# Autodesk Inventor assembly: Print_Assembly_H0_NEM363
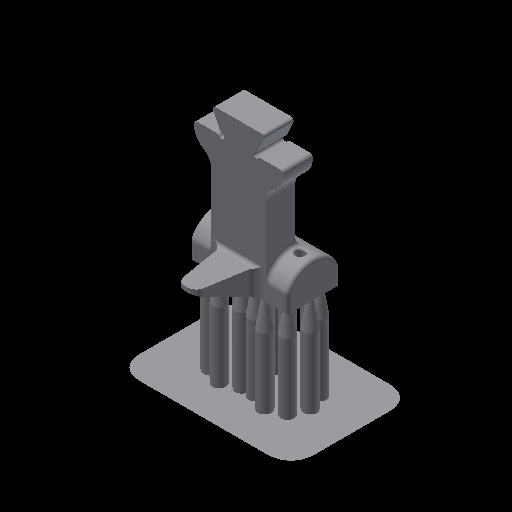
[picture p0: Inventor's stored thumbnail of the model, 512x512]
Saved by Autodesk Inventor 2026.2 (Build 302298010, 298A)
## iProperties
Manager: MANUTENÇÃO GUIFÕES - CP
Company: CP
Created: 2025-09-03
Part Number: Print_Assembly_H0_NEM363
Project: 0.00 0000/00
Checked By: PMFIGUEIREDO
Engr Approved By: JSSILVA
Description: NOME DA PEÇA/MONTAGEM
Document SubType Name: Assembly
Designer: TPMIRANDA
Engineer: ISO 2768 - m K
Authority: Nº DESENHO PELO QUAL FOI SUBSITUIDO
Stock Number: 00000-000
Title: UME 3400
Subject: CAIXA, INTERIOR, SUPORTE,
Author: TPMIRANDA
Keywords: Caixa de comentários. Substituir texto, ou eliminar.
Comments: UQE2300 UQE2400 UTE2240 UDD9630 CARRUAGENS SIMAFE CARRUAGENS CAF CARRUAGENS ARCO
Revision Number: Nº DESENHO QUE SUBSTITUI
## Documents named in this file (5)
- C:\Users\tpmiranda\OneDrive - Comboios de Portugal EPE\Engate CNMF\Montagem\Print_Assembly_H0_NEM363_Ø2.iam
- C:\Users\tpmiranda\OneDrive - Comboios de Portugal EPE\Engate CNMF\Montagem\Stand.ipt
- C:\Users\tpmiranda\OneDrive - Comboios de Portugal EPE\Engate CNMF\Montagem\Base h0.ipt
- C:\Users\tpmiranda\OneDrive - Comboios de Portugal EPE\Engate CNMF\Engates\Engate CNMF H0 NEM363 Ø2.ipt
- C:\Users\tpmiranda\OneDrive - Comboios de Portugal EPE\Engate CNMF\Engates\Engate CNMF H0 NEM363 Ø2\Engate CNMF NEM362-7.0.ipt
## Components (17 placed, 3 different names)
1. Base h0:1 — Alinhado:13, Alinhado:14, Alinhado:15
2. Engate CNMF NEM362-7.0:1 — Coincidente:1, Alinhado:4, Coincidente:2, Coincidente:9, Coincidente:10
3. Stand:1 — Alinhado:1, Coincidente:9, Alinhado:3, Coincidente:1
4. Stand:2 — Alinhado:5, Coincidente:10, Alinhado:7
5. Stand:3
6. Stand:4
7. Stand:5
8. Stand:6
9. Stand:7
10. Stand:8
11. Stand:9
12. Stand:10
13. Stand:11
14. Stand:12
15. Stand:13
16. Stand:14
17. Stand:15
## Component patterns: (2 elements), (7 elements, first: Stand:2), Componente de padrão 7:2 (7 elements)
## Relationships (12: Flush 8, Mate 4)
- Alinhado:1 [Flush]: Stand:1
- Coincidente:9 [Mate]: Engate CNMF NEM362-7.0:1 ↔ Stand:1
- Alinhado:3 [Flush]: Stand:1
- Coincidente:1 [Mate]: Engate CNMF NEM362-7.0:1 ↔ Stand:1
- Alinhado:4 [Flush]: Engate CNMF NEM362-7.0:1
- Coincidente:2 [Mate] (-3.5 mm): Engate CNMF NEM362-7.0:1
- Alinhado:5 [Flush] (2.6 mm): Stand:2
- Coincidente:10 [Mate]: Engate CNMF NEM362-7.0:1 ↔ Stand:2
- Alinhado:7 [Flush]: Stand:2
- Alinhado:13 [Flush]: Base h0:1
- Alinhado:14 [Flush]: Base h0:1
- Alinhado:15 [Flush] (-3.5 mm): Base h0:1
